# Autodesk Inventor assembly: top_frame_assy
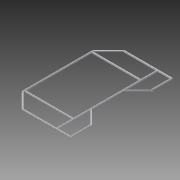
[picture p0: Inventor's stored thumbnail of the model, 180x180]
Saved by Autodesk Inventor 2015 (Build 190159000, 159)
## iProperties
Created: 2017-10-13
Part Number: top_frame_assy
Document SubType Name: Assembly
Designer: windows7
Author: windows7
## Documents named in this file (7)
- E:\COMPUTER_DESK\top_frame_assy.iam
- E:\COMPUTER_DESK\20_SERIES\20-2020.ipt
- E:\COMPUTER_DESK\20_SERIES\20-2020_1117.ipt
- E:\COMPUTER_DESK\20_SERIES\20-2020_508.ipt
- E:\COMPUTER_DESK\20_SERIES\20-2020_760.ipt
- E:\COMPUTER_DESK\20_SERIES\20-2020_320-45-parallel.ipt
- E:\computer_desk\20_Series\20-2020_726_MM.IPT
## Components (12 placed, 6 different names)
1. 20-2020:1 — Mate:33, Mate:34, Mate:35, Flush:14, Mate:36, Flush:15, Mate:37, Mate:38
2. 20-2020_1117:1 — Flush:15, Mate:37, Mate:38, Flush:21, Mate:52, Mate:53, Mate:72, Mate:73, Mate:74, Mate:75, Mate:76
3. 20-2020:2 — Flush:21, Mate:52, Mate:53, Mate:55, Mate:56, Mate:57
4. 20-2020_760:1 — Mate:44, Mate:45, Mate:55, Mate:56, Mate:57, Mate:58, Mate:65, Mate:66
5. 20-2020_760:2 — Mate:31, Mate:32, Mate:33, Mate:34, Mate:35, Flush:14, Mate:36
6. 20-2020_320-45-parallel:1 — Mate:44, Mate:45, Mate:46, Flush:18, Mate:47, Mate:58
7. 20-2020_320-45-parallel:3 — Mate:31, Mate:32, Flush:20, Mate:50, Mate:51
8. 20-2020_320-45-parallel:4 — Flush:20, Mate:50, Mate:51, Mate:67, Mate:68
9. 20-2020_320-45-parallel:5 — Mate:46, Flush:18, Mate:47
10. 20-2020_508:3 — Mate:65, Mate:66, Mate:67, Mate:68, Mate:77
11. 20-2020_726_MM:1 — Mate:72, Mate:73, Mate:77
12. 20-2020_726_MM:2 — Mate:74, Mate:75, Mate:76
## Relationships (35: Mate 30, Flush 5)
- Mate:31: 20-2020_760:2 ↔ 20-2020_320-45-parallel:3
- Mate:32: 20-2020_760:2 ↔ 20-2020_320-45-parallel:3
- Mate:33: 20-2020:1 ↔ 20-2020_760:2
- Mate:34: 20-2020:1 ↔ 20-2020_760:2
- Mate:35: 20-2020:1 ↔ 20-2020_760:2
- Flush:14: 20-2020:1 ↔ 20-2020_760:2
- Mate:36: 20-2020:1 ↔ 20-2020_760:2
- Flush:15: 20-2020:1 ↔ 20-2020_1117:1
- Mate:37: 20-2020:1 ↔ 20-2020_1117:1
- Mate:38: 20-2020:1 ↔ 20-2020_1117:1
- Mate:44: 20-2020_760:1 ↔ 20-2020_320-45-parallel:1
- Mate:45: 20-2020_760:1 ↔ 20-2020_320-45-parallel:1
- Mate:46: 20-2020_320-45-parallel:1 ↔ 20-2020_320-45-parallel:5
- Flush:18: 20-2020_320-45-parallel:1 ↔ 20-2020_320-45-parallel:5
- Mate:47: 20-2020_320-45-parallel:1 ↔ 20-2020_320-45-parallel:5
- Flush:20: 20-2020_320-45-parallel:3 ↔ 20-2020_320-45-parallel:4
- Mate:50: 20-2020_320-45-parallel:3 ↔ 20-2020_320-45-parallel:4
- Mate:51: 20-2020_320-45-parallel:3 ↔ 20-2020_320-45-parallel:4
- Flush:21: 20-2020_1117:1 ↔ 20-2020:2
- Mate:52: 20-2020_1117:1 ↔ 20-2020:2
- Mate:53: 20-2020_1117:1 ↔ 20-2020:2
- Mate:55: 20-2020:2 ↔ 20-2020_760:1
- Mate:56: 20-2020:2 ↔ 20-2020_760:1
- Mate:57: 20-2020:2 ↔ 20-2020_760:1
- Mate:58: 20-2020_760:1 ↔ 20-2020_320-45-parallel:1
- Mate:65: 20-2020_760:1 ↔ 20-2020_508:3
- Mate:66: 20-2020_760:1 ↔ 20-2020_508:3
- Mate:67: 20-2020_320-45-parallel:4 ↔ 20-2020_508:3
- Mate:68: 20-2020_320-45-parallel:4 ↔ 20-2020_508:3
- Mate:72: 20-2020_1117:1 ↔ 20-2020_726_MM:1
- Mate:73: 20-2020_1117:1 ↔ 20-2020_726_MM:1
- Mate:74: 20-2020_1117:1 ↔ 20-2020_726_MM:2
- Mate:75: 20-2020_1117:1 ↔ 20-2020_726_MM:2
- Mate:76: 20-2020_1117:1 ↔ 20-2020_726_MM:2
- Mate:77: 20-2020_508:3 ↔ 20-2020_726_MM:1
